# Autodesk Inventor assembly: 2axisRotator
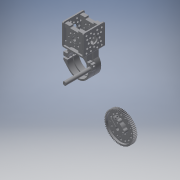
[picture p0: Inventor's stored thumbnail of the model, 180x180]
Saved by Autodesk Inventor 2018 (Build 220112000, 112)
## iProperties
Created: 2017-10-12
Part Number: 2axisRotator
Document SubType Name: Assembly
Designer: ball
Author: ball
## Documents named in this file (8)
- C:\FTC\2017 Robot\TestInventor\2axisRotator.iam
- C:\FTC\PTC Creo\Actobotics\585 parts\585440.ipt
- C:\FTC\PTC Creo\Actobotics\535 parts\535130 assembly.ipt
- C:\FTC\PTC Creo\Actobotics\634 parts\634068.ipt
- C:\FTC\PTC Creo\Actobotics\555 parts\555116.ipt
- C:\FTC\PTC Creo\Actobotics\625 parts\625102.ipt
- C:\FTC\PTC Creo\Actobotics\615 parts\615194.ipt
- C:\FTC\PTC Creo\Actobotics\545 parts\545619 assembly.ipt
## Components (9 placed, 7 different names)
1. 585440:1 — Insert:1, Insert:2, Insert:3, Insert:4, Insert:5, Insert:7, Insert:9, Insert:10
2. 535130 assembly:1 — Insert:1, Insert:2
3. 535130 assembly:2 — Insert:3, Insert:4
4. 634068:1 — Flush:1
5. 555116:1 — Insert:9, Insert:10
6. 555116:2 — Insert:5, Insert:7
7. 625102:1 — Flush:1
8. 615194:1 — Insert:8, Mate:1
9. 545619 assembly:2 — Insert:8, Mate:1
## Relationships (11: Insert 9, Flush 1, Mate 1)
- Insert:1: 585440:1 ↔ 535130 assembly:1
- Insert:2: 585440:1 ↔ 535130 assembly:1
- Insert:3: 585440:1 ↔ 535130 assembly:2
- Insert:4: 585440:1 ↔ 535130 assembly:2
- Insert:5: 585440:1 ↔ 555116:2
- Insert:7: 585440:1 ↔ 555116:2
- Flush:1: 634068:1 ↔ 625102:1
- Insert:8: 615194:1 ↔ 545619 assembly:2
- Insert:9: 585440:1 ↔ 555116:1
- Insert:10: 585440:1 ↔ 555116:1
- Mate:1: 615194:1 ↔ 545619 assembly:2
